# Autodesk Inventor assembly: ASY Beshkino main
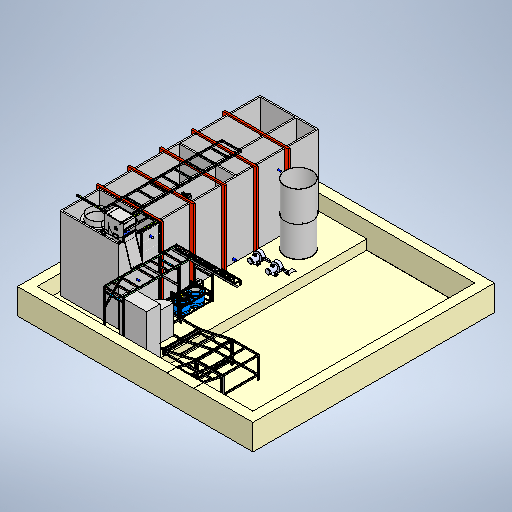
[picture p0: Inventor's stored thumbnail of the model, 512x512]
Saved by Autodesk Inventor 2025.1 (Build 291241020, 241B)
## iProperties
Created: 2024-08-27
Part Number: ASY Beshkino main
Document SubType Name: Assembly
Designer: DELL
Author: DELL
## Documents named in this file (23)
- C:\Users\user\YandexDisk-badmisterfox\домашниий пк\Inventor\BSH_Beshkino_bio_tank\ASY Beshkino main.iam
- C:\Users\user\YandexDisk-badmisterfox\домашниий пк\Inventor\BSH_Beshkino_bio_tank\BSH 0 foudation.ipt
- C:\Users\user\YandexDisk-badmisterfox\домашниий пк\Inventor\BSH_Beshkino_bio_tank\ASY Beshkino_bio_tank.iam
- C:\Users\user\YandexDisk-badmisterfox\домашниий пк\Inventor\BSH_Beshkino_bio_tank\ASY Trommel.iam
- C:\Users\user\YandexDisk-badmisterfox\домашниий пк\Inventor\BSH_Beshkino_bio_tank\3d party\RXm3 assieme dimensionale mag2018.ipt
- C:\Users\user\YandexDisk-badmisterfox\домашниий пк\Inventor\BSH_Beshkino_bio_tank\3d party\motor-reductor NMRV040\motor-reductor NMRV040.iam
- C:\Users\user\YandexDisk-badmisterfox\домашниий пк\Inventor\BSH_Beshkino_bio_tank\BSH 01 foam filter.ipt
- C:\Users\user\YandexDisk-badmisterfox\домашниий пк\Inventor\BSH_Beshkino_bio_tank\BSH 01 bag.ipt
- C:\Users\user\YandexDisk-badmisterfox\домашниий пк\Inventor\BSH_Beshkino_bio_tank\BSH 03 upstairs.ipt
- C:\Users\user\YandexDisk-badmisterfox\домашниий пк\Inventor\BSH_Beshkino_bio_tank\лестница\Перегородка\ASY NDM 11.0 перегородка.iam
- C:\Users\user\YandexDisk-badmisterfox\домашниий пк\Inventor\BSH_Beshkino_bio_tank\Конструкция.iam
- C:\Users\user\YandexDisk-badmisterfox\домашниий пк\Inventor\BSH_Beshkino_bio_tank\ASY BSH 500 cap.iam
- C:\Users\user\YandexDisk-badmisterfox\домашниий пк\Inventor\BSH_Beshkino_bio_tank\ASY 080 barrel.iam
- C:\Users\user\YandexDisk-badmisterfox\домашниий пк\Inventor\BSH_Beshkino_bio_tank\BSH 600 Tank dummy.ipt
- C:\Users\user\YandexDisk-badmisterfox\домашниий пк\Inventor\BSH_Beshkino_bio_tank\3d party\airpump\EVL 64-41.ipt
- C:\Users\user\YandexDisk-badmisterfox\домашниий пк\Inventor\BSH_Beshkino_bio_tank\ISO 12633-2 - 50x50x3 - 1500.ipt
- C:\Users\user\YandexDisk-badmisterfox\домашниий пк\Inventor\BSH_Beshkino_bio_tank\ISO 12633-2 - 20x20x2 - 2000.ipt
- C:\Users\user\YandexDisk-badmisterfox\домашниий пк\Inventor\BSH_Beshkino_bio_tank\Настил большой.iam
- C:\Users\user\YandexDisk-badmisterfox\домашниий пк\Inventor\BSH_Beshkino_bio_tank\Настил маленький.iam
- C:\Users\user\YandexDisk-badmisterfox\домашниий пк\Inventor\BSH_Beshkino_bio_tank\Лестница вертикальная.iam
- C:\Users\user\YandexDisk-badmisterfox\домашниий пк\Inventor\BSH_Beshkino_bio_tank\Пандус.iam
- C:\Users\user\YandexDisk-badmisterfox\домашниий пк\Inventor\BSH_Beshkino_bio_tank\ASY BSH 610 reagent dosator.iam
- C:\Users\user\YandexDisk-badmisterfox\домашниий пк\Inventor\BSH_Beshkino_bio_tank\BSH pollar 5.ipt
## Components (25 placed, 22 different names)
1. BSH 0 foudation:1 — Mate:1, Mate:2, Mate:3, Mate:4, Flush:2, Flush:3, Flush:4, Flush:5, Mate:10, Mate:12, Mate:13, Mate:14, Mate:15, Mate:18, Mate:23
2. ASY Beshkino_bio_tank:1 [sub-assembly] — Mate:2, Mate:3, Mate:4, Mate:5, Mate:6
3. ASY Trommel:1 [sub-assembly] — Mate:9, Flush:6
4. RXm3 assieme dimensionale mag2018:1 — Mate:5
5. RXm3 assieme dimensionale mag2018:2 — Mate:6
6. motor-reductor NMRV040:1 [sub-assembly]
7. BSH 01 foam filter:1 — Flush:2, Rigid:1
8. BSH 01 bag:1 — Flush:3, Mate:14
9. BSH 03 upstairs:1 — Flush:4
10. ASY NDM 11.0 перегородка:1 [sub-assembly]
11. Конструкция:1 [sub-assembly] — Mate:10, Mate:11
12. ASY BSH 500 cap:1 [sub-assembly] — Rigid:1
13. ASY 080 barrel:1 [sub-assembly] — Mate:8
14. BSH 600 Tank dummy:1 — Flush:5, Mate:8, Mate:9, Mate:11, Mate:12, Mate:13, Flush:6, Mate:19, Flush:8, Flush:10, Mate:21, Flush:11, Flush:12
15. EVL 64-41:1 — Mate:15
16. EVL 64-41:2 — Mate:18
17. ISO 12633-2 - 50x50x3 - 1500:1 — Mate:19, Flush:8, Rigid:2, Flush:10
18. ISO 12633-2 - 50x50x3 - 1500:2 — Rigid:2, Mate:20, Flush:9
19. ISO 12633-2 - 20x20x2 - 2000:1 — Mate:20, Flush:9
20. Настил большой:1 [sub-assembly] — Mate:21, Flush:11, Rigid:3
21. Настил маленький:1 [sub-assembly] — Rigid:3, Flush:12, Rigid:4
22. Лестница вертикальная:1 [sub-assembly] — Rigid:4
23. Пандус:1 [sub-assembly]
24. ASY BSH 610 reagent dosator:1 [sub-assembly]
25. BSH pollar 5:1 — Mate:23
## Relationships (35: Mate 20, Flush 11, WeldJoint 4)
- Mate:1: BSH 0 foudation:1
- Mate:2: BSH 0 foudation:1 ↔ ASY Beshkino_bio_tank:1
- Mate:3 (100 mm): BSH 0 foudation:1 ↔ ASY Beshkino_bio_tank:1
- Mate:4 (200 mm): BSH 0 foudation:1 ↔ ASY Beshkino_bio_tank:1
- Mate:5: ASY Beshkino_bio_tank:1 ↔ RXm3 assieme dimensionale mag2018:1
- Mate:6: ASY Beshkino_bio_tank:1 ↔ RXm3 assieme dimensionale mag2018:2
- Flush:2: BSH 0 foudation:1 ↔ BSH 01 foam filter:1
- Flush:3: BSH 0 foudation:1 ↔ BSH 01 bag:1
- Flush:4: BSH 0 foudation:1 ↔ BSH 03 upstairs:1
- Flush:5: BSH 0 foudation:1 ↔ BSH 600 Tank dummy:1
- Mate:8: ASY 080 barrel:1 ↔ BSH 600 Tank dummy:1
- Mate:9 (50 mm): ASY Trommel:1 ↔ BSH 600 Tank dummy:1
- Mate:10: BSH 0 foudation:1 ↔ Конструкция:1
- Mate:11 (10 mm): Конструкция:1 ↔ BSH 600 Tank dummy:1
- Mate:12: BSH 0 foudation:1 ↔ BSH 600 Tank dummy:1
- Mate:13 (100 mm): BSH 0 foudation:1 ↔ BSH 600 Tank dummy:1
- Flush:6 (-100 mm): ASY Trommel:1 ↔ BSH 600 Tank dummy:1
- Mate:14 (100 mm): BSH 0 foudation:1 ↔ BSH 01 bag:1
- Mate:15: BSH 0 foudation:1 ↔ EVL 64-41:1
- Mate:18: BSH 0 foudation:1 ↔ EVL 64-41:2
- Rigid:1 [WeldJoint]: BSH 01 foam filter:1 ↔ ASY BSH 500 cap:1
- Mate:19: BSH 600 Tank dummy:1 ↔ ISO 12633-2 - 50x50x3 - 1500:1
- Flush:8: BSH 600 Tank dummy:1 ↔ ISO 12633-2 - 50x50x3 - 1500:1
- Rigid:2 [WeldJoint] (400 mm): ISO 12633-2 - 50x50x3 - 1500:1 ↔ ISO 12633-2 - 50x50x3 - 1500:2
- Mate:20: ISO 12633-2 - 50x50x3 - 1500:2 ↔ ISO 12633-2 - 20x20x2 - 2000:1
- Flush:9: ISO 12633-2 - 50x50x3 - 1500:2 ↔ ISO 12633-2 - 20x20x2 - 2000:1
- Flush:10: BSH 600 Tank dummy:1 ↔ ISO 12633-2 - 50x50x3 - 1500:1
- Mate:21: BSH 600 Tank dummy:1 ↔ Настил большой:1
- Flush:11 (-150 mm): BSH 600 Tank dummy:1 ↔ Настил большой:1
- Rigid:3 [WeldJoint]: Настил большой:1 ↔ Настил маленький:1
- Flush:12: BSH 600 Tank dummy:1 ↔ Настил маленький:1
- Rigid:4 [WeldJoint]: Настил маленький:1 ↔ Лестница вертикальная:1
- [Mate]: BSH 0 foudation:1 ↔ Пандус:1
- [Flush]: BSH 0 foudation:1 ↔ ASY BSH 610 reagent dosator:1
- Mate:23: BSH 0 foudation:1 ↔ BSH pollar 5:1
